# Autodesk Inventor assembly: Main Assem
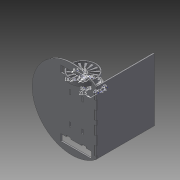
[picture p0: Inventor's stored thumbnail of the model, 180x180]
Saved by Autodesk Inventor 2015 (Build 190159000, 159)
## iProperties
Created: 2014-07-26
Part Number: Main Assem
Document SubType Name: Assembly
Designer: karl
Author: karl
## Documents named in this file (7)
- C:\Users\karl\Documents\GitHub\QUT-Robotics-Club----Sumo-Bots\Body\Main frame\Main Assem.iam
- C:\Users\karl\Documents\GitHub\QUT-Robotics-Club----Sumo-Bots\Body\Main frame\BasePlate.ipt
- C:\Users\karl\Documents\GitHub\QUT-Robotics-Club----Sumo-Bots\Body\Main frame\Motor mount.ipt
- C:\Users\karl\Documents\GitHub\QUT-Robotics-Club----Sumo-Bots\Body\Main frame\Wheel.ipt
- C:\Users\karl\Documents\GitHub\QUT-Robotics-Club----Sumo-Bots\Body\Main frame\Motor side.ipt
- C:\Users\karl\Documents\GitHub\QUT-Robotics-Club----Sumo-Bots\Body\Main frame\frount plate.ipt
- C:\Users\karl\Documents\GitHub\QUT-Robotics-Club----Sumo-Bots\Body\Main frame\Mid Plate.ipt
## Components (7 placed, 6 different names)
1. BasePlate:1 — Flush:1, Mate:1, Flush:2, Mate:5, Mate:7, Flush:6, Mate:8
2. Motor mount:1 — Flush:1, Mate:1, Flush:2, Mate:2, Mate:3, Mate:4, Flush:3, Flush:4, Mate:6, Flush:7
3. Wheel:1 — Mate:2, Mate:3
4. Motor side:1 — Mate:4, Mate:5, Flush:3, Flush:5, Flush:8
5. Motor side:2 — Flush:4, Flush:5, Mate:6
6. frount plate:1 — Mate:7, Flush:6, Mate:8, Mate:9
7. Mid Plate:1 — Flush:7, Mate:9, Flush:8
## Relationships (17: Mate 9, Flush 8)
- Flush:1: BasePlate:1 ↔ Motor mount:1
- Mate:1: BasePlate:1 ↔ Motor mount:1
- Flush:2: BasePlate:1 ↔ Motor mount:1
- Mate:2: Motor mount:1 ↔ Wheel:1
- Mate:3 (3 mm): Motor mount:1 ↔ Wheel:1
- Mate:4: Motor mount:1 ↔ Motor side:1
- Mate:5: BasePlate:1 ↔ Motor side:1
- Flush:3: Motor mount:1 ↔ Motor side:1
- Flush:4: Motor mount:1 ↔ Motor side:2
- Flush:5: Motor side:1 ↔ Motor side:2
- Mate:6: Motor mount:1 ↔ Motor side:2
- Mate:7: BasePlate:1 ↔ frount plate:1
- Flush:6: BasePlate:1 ↔ frount plate:1
- Mate:8: BasePlate:1 ↔ frount plate:1
- Flush:7: Motor mount:1 ↔ Mid Plate:1
- Mate:9: frount plate:1 ↔ Mid Plate:1
- Flush:8: Motor side:1 ↔ Mid Plate:1
